# Autodesk Inventor assembly: 00_ESP3-CAM_wSpacer
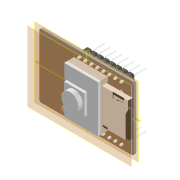
[picture p0: Inventor's stored thumbnail of the model, 180x180]
Saved by Autodesk Inventor 2022 (Build 260153000, 153)
## iProperties
Created: 2022-08-19
Part Number: 00_ESP3-CAM_wSpacer
Document SubType Name: Assembly
Designer: UC2
Author: UC2
## Documents named in this file (3)
- C:\Users\UC2\Documents\GitHub\Matchboxscope\INVENTOR\00_ESP3-CAM_wSpacer.iam
- C:\Users\UC2\Documents\GitHub\Matchboxscope\INVENTOR\00_ESP3-CAM.iam
- C:\Users\UC2\Documents\GitHub\Matchboxscope\INVENTOR\00_ESP32_OmnivisionCameraModule.ipt
## Components (2 placed, 2 different names)
1. 00_ESP3-CAM:1 [sub-assembly] — Fluchtend:1, Fluchtend:2
2. 00_ESP32_OmnivisionCameraModule:1 — Fluchtend:1, Fluchtend:2
## Relationships (2: Flush 2)
- Fluchtend:1 [Flush]: 00_ESP3-CAM:1 ↔ 00_ESP32_OmnivisionCameraModule:1
- Fluchtend:2 [Flush] (2.9972 mm): 00_ESP3-CAM:1 ↔ 00_ESP32_OmnivisionCameraModule:1
